# Autodesk Inventor assembly: 組み合わせギア_0.5-100_SSY1_15
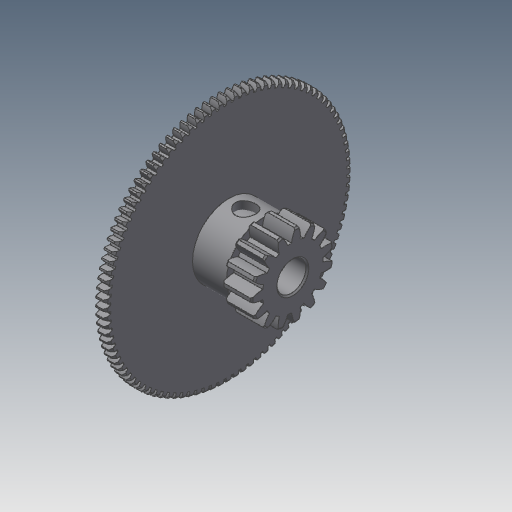
[picture p0: Inventor's stored thumbnail of the model, 512x512]
Saved by Autodesk Inventor 2019 (Build 230136000, 136)
## iProperties
Created: 2020-10-25
Part Number: 組み合わせギア_0.5-100_SSY1_15
Material: 一般
Document SubType Name: Assembly
Designer: zhept
Mass: 6.1641 g
Surface Area: 63.7341 cm^2
Volume: 6.1641 cm^3
Density: 1 g/cm^3
Author: zhept
## iProperties of the stored document SS0.5-100A_On.ipt
Company: CADENAS
Created: 2020-09-08
Part Number: SS0.5-100A_On
Material: 一般
Description: STEP AP203
Document SubType Name: Modeling
Designer: zhept
Density: 1 g/cm^3
Appearance: 既定
Mass: 13.3283 g
Surface Area: 62.7451 cm^2
Volume: 13.3283 cm^3
Sending System: PARTsolutions
Title: p:/temp/worker_5/temp/exporttempdir_3536_1079_4FBt6/format_0/SS0.5-100A_On.stp
Author: License CC BY-ND 4.0
Revision Number: NONE
## iProperties of the stored document SSY1-15_On.ipt
Company: CADENAS
Created: 2020-10-25
Part Number: SSY1-15_On
Material: 一般
Description: STEP AP203
Document SubType Name: Modeling
Designer: zhept
Density: 1 g/cm^3
Appearance: 既定
Mass: 1.53173 g
Surface Area: 13.9391 cm^2
Volume: 1.53173 cm^3
Sending System: PARTsolutions
Title: p:/temp/worker_8/temp/exporttempdir_1868_509_Byv7i/format_0/SSY1-15_On.stp
Author: License CC BY-ND 4.0
Revision Number: NONE
## Documents named in this file (5)
- C:\Users\zhept\OneDrive\大学\rrst\足回り2020\上層部v2\組み合わせギア_0.5-100_SSY1_15.iam
- **C:\Users\zhept\OneDrive\大学\rrst\足回り2020\上層部v2\組み合わせギア_0.5-100_SSY1_15.iam*LocalDocs*xNdblixwh0p24e2oh4j5etyjgBf*SSY1-15_On.ipt
- **C:\Users\zhept\OneDrive\大学\rrst\足回り2020\上層部v2\組み合わせギア_0.5-100_SSY1_15.iam*LocalDocs*xHqrp45o0YpyxetciIxghoswjPc*SS0.5-100A_On.ipt
- C:\Users\zhept\OneDrive\大学\rrst\足回り2020\上層部v2\SSY1-15_On.stp
- C:\Users\zhept\OneDrive\大学\rrst\足回り2020\上層部v2\SS0.5-100A_On.stp
## Components (2 placed, 2 different names)
1. SSY1-15_On:1 — 回転:1
2. SS0.5-100A_On:1 — 回転:1
## Relationships (1: RevoluteJoint 1)
- 回転:1 [RevoluteJoint]: SSY1-15_On:1 ↔ SS0.5-100A_On:1
